# Autodesk Inventor assembly: HDPE Body
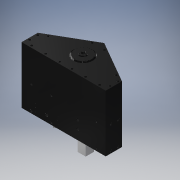
[picture p0: Inventor's stored thumbnail of the model, 180x180]
Saved by Autodesk Inventor 2017 (Build 210142000, 142)
## iProperties
Created: 2019-05-20
Part Number: HDPE Body
Document SubType Name: Assembly
Designer: Dell
Mass: 14814 g
Surface Area: 22717.5 cm^2
Volume: 13790.6 cm^3
Density: 1.07421 g/cm^3
Author: Dell
## Documents named in this file (11)
- C:\Users\Dell\Documents\GitHub\tr2\Body\HDPE Body.iam
- C:\Users\Dell\Documents\GitHub\tr2\Body\HB01.ipt
- C:\Users\Dell\Documents\GitHub\tr2\Body\HB02.ipt
- C:\Users\Dell\Documents\GitHub\tr2\Body\HB03.ipt
- C:\Users\Dell\Documents\GitHub\tr2\Body\HB04.ipt
- C:\Users\Dell\Documents\GitHub\tr2\Body\HB05.ipt
- C:\Users\Dell\Documents\GitHub\tr2\Body\HB01b.ipt
- C:\Users\Dell\Documents\GitHub\tr2\Body\ST22.ipt
- C:\Users\Dell\Documents\GitHub\tr2\Body\HB05b.ipt
- C:\Users\Dell\Documents\GitHub\tr2\Actuator 1.3\Actuator 1.3.iam
- C:\Users\Dell\Documents\GitHub\tr2\Body\HB02b.ipt
## Components (12 placed, 10 different names)
1. HB01:1 — Mate:1, Flush:1, Mate:2, Flush:6, Mate:8, Mate:14, Flush:11, Mate:35, Mate:64, Mate:65, Mate:66, Mate:67, Mate:87, Mate:88
2. HB02:1 — Mate:1, Flush:1, Mate:2, Mate:12, Flush:9, Mate:43, Mate:47, Mate:50, Mate:72, Mate:73, Mate:83
3. HB03:1 — Flush:6, Flush:7, Mate:32, Mate:33, Mate:38, Mate:74, Mate:75, Mate:76, Mate:77, Mate:78, Mate:79, Mate:80, Mate:81, Mate:82, Mate:89, Mate:90, Mate:91, Mate:92, Mate:93, Mate:94
4. HB04:1 — Mate:8, Flush:7, Flush:9, Mate:18, Flush:10, Mate:32, Mate:44, Flush:12, Mate:83, Mate:84, Mate:85, Mate:86, Mate:87, Mate:88, Mate:89, Mate:90, Mate:91, Mate:92, Mate:93, Mate:94
5. HB05:2 — Mate:12, Mate:14, Mate:46, Mate:49, Mate:50, Mate:52, Mate:53, Mate:57, Mate:58, Mate:60, Mate:61, Mate:66, Mate:67, Mate:68, Mate:69, Mate:74, Mate:75, Mate:77, Mate:78
6. HB01b:1 — Mate:18, Flush:10, Flush:11, Mate:45, Mate:46, Mate:62, Mate:63, Mate:68, Mate:69, Mate:86
7. HB05b:1 — Mate:33, Mate:35, Mate:38, Mate:40, Mate:41, Mate:42, Mate:47, Mate:48, Mate:56, Mate:59, Mate:62, Mate:63, Mate:64, Mate:65, Mate:76, Mate:79, Mate:80
8. ST22:1 — Mate:59, Mate:60, Mate:61, Mate:72, Mate:73
9. ST22:2 — Mate:56, Mate:57, Mate:58, Mate:81, Mate:82
10. ST22:3 — Mate:52, Mate:53, Mate:54, Mate:55, Mate:70, Mate:71
11. Actuator 1.3:1 [sub-assembly] — Mate:40, Mate:41, Mate:42
12. HB02b:1 — Mate:43, Mate:44, Mate:45, Flush:12, Mate:48, Mate:49, Mate:54, Mate:55, Mate:70, Mate:71, Mate:84, Mate:85
## Relationships (71: Mate 64, Flush 7)
- Mate:1: HB01:1 ↔ HB02:1
- Flush:1: HB01:1 ↔ HB02:1
- Mate:2: HB01:1 ↔ HB02:1
- Flush:6: HB01:1 ↔ HB03:1
- Mate:8: HB01:1 ↔ HB04:1
- Flush:7: HB03:1 ↔ HB04:1
- Mate:12: HB02:1 ↔ HB05:2
- Mate:14: HB01:1 ↔ HB05:2
- Flush:9: HB02:1 ↔ HB04:1
- Mate:18: HB04:1 ↔ HB01b:1
- Flush:10: HB04:1 ↔ HB01b:1
- Flush:11: HB01:1 ↔ HB01b:1
- Mate:32: HB03:1 ↔ HB04:1
- Mate:33: HB03:1 ↔ HB05b:1
- Mate:35: HB01:1 ↔ HB05b:1
- Mate:38: HB03:1 ↔ HB05b:1
- Mate:40: HB05b:1 ↔ Actuator 1.3:1
- Mate:41: HB05b:1 ↔ Actuator 1.3:1
- Mate:42: HB05b:1 ↔ Actuator 1.3:1
- Mate:43: HB02:1 ↔ HB02b:1
- Mate:44: HB04:1 ↔ HB02b:1
- Mate:45: HB01b:1 ↔ HB02b:1
- Flush:12: HB04:1 ↔ HB02b:1
- Mate:46: HB05:2 ↔ HB01b:1
- Mate:47: HB02:1 ↔ HB05b:1
- Mate:48: HB05b:1 ↔ HB02b:1
- Mate:49: HB05:2 ↔ HB02b:1
- Mate:50: HB02:1 ↔ HB05:2
- Mate:52: HB05:2 ↔ ST22:3
- Mate:53: HB05:2 ↔ ST22:3
- Mate:54: ST22:3 ↔ HB02b:1
- Mate:55: ST22:3 ↔ HB02b:1
- Mate:56: HB05b:1 ↔ ST22:2
- Mate:57: HB05:2 ↔ ST22:2
- Mate:58: HB05:2 ↔ ST22:2
- Mate:59: HB05b:1 ↔ ST22:1
- Mate:60: HB05:2 ↔ ST22:1
- Mate:61: HB05:2 ↔ ST22:1
- Mate:62: HB01b:1 ↔ HB05b:1
- Mate:63: HB01b:1 ↔ HB05b:1
- Mate:64: HB01:1 ↔ HB05b:1
- Mate:65: HB01:1 ↔ HB05b:1
- Mate:66: HB01:1 ↔ HB05:2
- Mate:67: HB01:1 ↔ HB05:2
- Mate:68: HB05:2 ↔ HB01b:1
- Mate:69: HB05:2 ↔ HB01b:1
- Mate:70: ST22:3 ↔ HB02b:1
- Mate:71: ST22:3 ↔ HB02b:1
- Mate:72: HB02:1 ↔ ST22:1
- Mate:73: HB02:1 ↔ ST22:1
- Mate:74: HB03:1 ↔ HB05:2
- Mate:75: HB03:1 ↔ HB05:2
- Mate:76: HB03:1 ↔ HB05b:1
- Mate:77: HB03:1 ↔ HB05:2
- Mate:78: HB03:1 ↔ HB05:2
- Mate:79: HB03:1 ↔ HB05b:1
- Mate:80: HB03:1 ↔ HB05b:1
- Mate:81: HB03:1 ↔ ST22:2
- Mate:82: HB03:1 ↔ ST22:2
- Mate:83: HB02:1 ↔ HB04:1
- Mate:84: HB04:1 ↔ HB02b:1
- Mate:85: HB04:1 ↔ HB02b:1
- Mate:86: HB04:1 ↔ HB01b:1
- Mate:87: HB01:1 ↔ HB04:1
- Mate:88: HB01:1 ↔ HB04:1
- Mate:89: HB03:1 ↔ HB04:1
- Mate:90: HB03:1 ↔ HB04:1
- Mate:91: HB03:1 ↔ HB04:1
- Mate:92: HB03:1 ↔ HB04:1
- Mate:93: HB03:1 ↔ HB04:1
- Mate:94: HB03:1 ↔ HB04:1
